# Autodesk Inventor assembly: Test Section
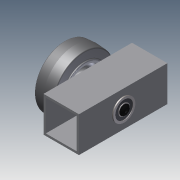
[picture p0: Inventor's stored thumbnail of the model, 180x180]
Saved by Autodesk Inventor 2014 SP1 (Build 180222100, 222)
## iProperties
Created: 2013-11-28
Part Number: Test Section
Document SubType Name: Assembly
Designer: Rauhul Varma
Author: Rauhul Varma
## Documents named in this file (8)
- C:\Users\Rauhul Varma\Desktop\2014 Base\Test Section.iam
- C:\Users\Rauhul Varma\Desktop\2014 Base\Box Beam.ipt
- C:\Users\Rauhul Varma\Desktop\2014 Base\22T 5mm GT2 Pulley.ipt
- C:\Users\Rauhul Varma\Desktop\2014 Base\FR8-2RS Bearing.ipt
- C:\Users\Rauhul Varma\Desktop\2014 Base\Live Axle.ipt
- C:\Users\Rauhul Varma\Desktop\2014 Base\FBHCS .25-20 .5000 Long.ipt
- C:\Users\Rauhul Varma\Desktop\2014 Base\Colson Hub.ipt
- C:\Users\Rauhul Varma\Desktop\2014 Base\3.5 in by 1.25 in Colson Wheel.ipt
## Components (9 placed, 7 different names)
1. Box Beam:1 — Mate:1, Mate:2, Mate:3, Mate:4, Mate:5
2. 22T 5mm GT2 Pulley:1 — Mate:1, Mate:6, Mate:12
3. FR8-2RS Bearing:1 — Mate:4, Mate:5, Mate:6, Mate:7, Mate:15
4. FR8-2RS Bearing:2 — Mate:2, Mate:3, Flush:1
5. Live Axle:1 — Mate:7, Flush:1, Mate:8, Mate:9, Mate:10, Mate:11, Mate:12, Mate:13, Mate:14
6. FBHCS .25-20 .5000 Long:1 — Mate:8, Mate:9
7. FBHCS .25-20 .5000 Long:2 — Mate:10, Mate:11
8. Colson Hub:1 — Mate:13, Mate:14, Mate:15, Mate:16, Mate:17
9. 3.5 in by 1.25 in Colson Wheel:1 — Mate:16, Mate:17
## Relationships (18: Mate 17, Flush 1)
- Mate:1: Box Beam:1 ↔ 22T 5mm GT2 Pulley:1
- Mate:2: Box Beam:1 ↔ FR8-2RS Bearing:2
- Mate:3: Box Beam:1 ↔ FR8-2RS Bearing:2
- Mate:4: Box Beam:1 ↔ FR8-2RS Bearing:1
- Mate:5: Box Beam:1 ↔ FR8-2RS Bearing:1
- Mate:6: 22T 5mm GT2 Pulley:1 ↔ FR8-2RS Bearing:1
- Mate:7: FR8-2RS Bearing:1 ↔ Live Axle:1
- Flush:1: FR8-2RS Bearing:2 ↔ Live Axle:1
- Mate:8: Live Axle:1 ↔ FBHCS .25-20 .5000 Long:1
- Mate:9: Live Axle:1 ↔ FBHCS .25-20 .5000 Long:1
- Mate:10: Live Axle:1 ↔ FBHCS .25-20 .5000 Long:2
- Mate:11: Live Axle:1 ↔ FBHCS .25-20 .5000 Long:2
- Mate:12: 22T 5mm GT2 Pulley:1 ↔ Live Axle:1
- Mate:13: Live Axle:1 ↔ Colson Hub:1
- Mate:14: Live Axle:1 ↔ Colson Hub:1
- Mate:15: FR8-2RS Bearing:1 ↔ Colson Hub:1
- Mate:16: Colson Hub:1 ↔ 3.5 in by 1.25 in Colson Wheel:1
- Mate:17: Colson Hub:1 ↔ 3.5 in by 1.25 in Colson Wheel:1
